# Autodesk Inventor assembly: VerticalParking
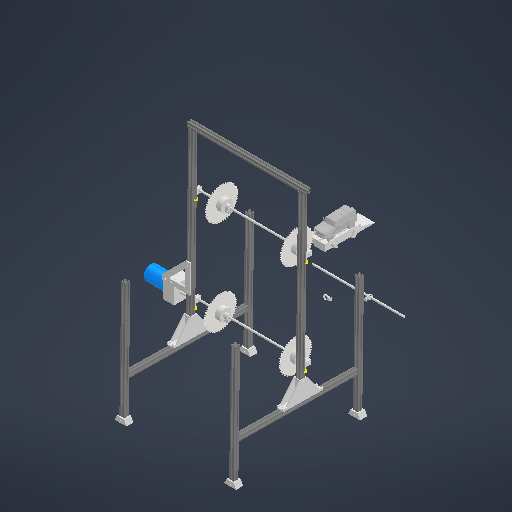
[picture p0: Inventor's stored thumbnail of the model, 512x512]
Saved by Autodesk Inventor 2026.1 (Build 301233020, 233B)
## iProperties
Created: 2025-12-07
Part Number: VerticalParking
Document SubType Name: Assembly
Designer: Tito Luyo Murata
Author: Tito Luyo Murata
## Documents named in this file (20)
- C:\work\verticalparking\diseno3d\VerticalParking.iam
- C:\work\verticalparking\diseno3d\01_Partes\soporte motor.ipt
- C:\work\verticalparking\diseno3d\01_Partes\Escuadra soporte motor.ipt
- C:\work\verticalparking\diseno3d\01_Partes\diseño piezas\motor_v02.ipt
- C:\work\verticalparking\diseno3d\01_Partes\Perfil_Aluminio_20x20x750.ipt
- C:\work\verticalparking\diseno3d\01_Partes\Perfil_Aluminio_20x20x500.ipt
- C:\work\verticalparking\diseno3d\01_Partes\base de soporte.ipt
- C:\work\verticalparking\diseno3d\01_Partes\SoportePrincipal.ipt
- C:\work\verticalparking\diseno3d\01_Partes\diseño piezas\soporte de eje de carril.ipt
- C:\work\verticalparking\diseno3d\01_Partes\diseño piezas\barrilla.ipt
- C:\work\verticalparking\diseno3d\01_Partes\diseño piezas\piñon.iam
- C:\work\verticalparking\diseno3d\01_Partes\SoporteEjePlato.ipt
- C:\work\verticalparking\diseno3d\01_Partes\SeguroRueda.ipt
- C:\work\verticalparking\diseno3d\01_Partes\RuedaDentada_v02.ipt
- C:\work\verticalparking\diseno3d\01_Partes\RuedaDentada_EjeFijo.ipt
- C:\work\verticalparking\diseno3d\01_Partes\Abrazadera.ipt
- C:\work\verticalparking\diseno3d\01_Partes\BaseCabina_v03.ipt
- C:\work\verticalparking\diseno3d\01_Partes\external\hammer_h3_v2\HermesH3v2.ipt
- C:\work\verticalparking\diseno3d\01_Partes\diseño piezas\barrilla_aluminio_385.ipt
- C:\work\verticalparking\diseno3d\01_Partes\AgarreColganteCabina_v02.ipt
## Components (55 placed, 19 different names)
1. soporte motor:1 — Mate:1, Mate:2, Mate:3, Mate:4, Mate:5, Mate:7
2. Escuadra soporte motor:1 — Mate:4, Mate:5, Mate:6, Mate:7, Flush:1, Flush:6
3. motor_v02:1 — Mate:1, Mate:2, Mate:3
4. Perfil_Aluminio_20x20x750:1 — Mate:9, Flush:3, Flush:5, Mate:16, Mate:17, Flush:16, Mate:18, Flush:17, Mate:29, Flush:21, Flush:23, Mate:32, Flush:26
5. Perfil_Aluminio_20x20x750:2 — Mate:6, Flush:1, Mate:8, Flush:2, Flush:4, Flush:6, Mate:14, Mate:15, Flush:15, Mate:19, Flush:19, Mate:30, Flush:22, Flush:24, Mate:33, Flush:27
6. Perfil_Aluminio_20x20x500:1 — Mate:8, Flush:2, Mate:9, Flush:3, Flush:4, Flush:5
7. Perfil_Aluminio_20x20x500:3 — Mate:10, Flush:7, Flush:8, Mate:11, Flush:9, Flush:10, Mate:18, Flush:17, Flush:18
8. Perfil_Aluminio_20x20x500:4 — Mate:11, Flush:9, Flush:10, Mate:26, Mate:27, Mate:28
9. Perfil_Aluminio_20x20x500:5 — Mate:12, Flush:11, Flush:12, Mate:20, Mate:21, Mate:22
10. Perfil_Aluminio_20x20x500:6 — Mate:13, Flush:13, Flush:14, Mate:23, Mate:24, Mate:25
11. Perfil_Aluminio_20x20x500:7 — Mate:10, Flush:7, Flush:8, Mate:51, Mate:52, Mate:53
12. Perfil_Aluminio_20x20x500:8 — Mate:12, Flush:11, Flush:12, Mate:13, Flush:13, Flush:14, Mate:19, Flush:19, Flush:20
13. base de soporte:1 — Mate:51, Mate:52, Mate:53
14. base de soporte:2 — Mate:23, Mate:24, Mate:25
15. base de soporte:3 — Mate:26, Mate:27, Mate:28
16. base de soporte:4 — Mate:20, Mate:21, Mate:22
17. SoportePrincipal:1 — Mate:16, Mate:17, Flush:16, Flush:18
18. SoportePrincipal:2 — Mate:14, Mate:15, Flush:15, Flush:20, Mate:74
19. soporte de eje de carril:1 — Mate:29, Flush:21, Flush:23, Mate:31, Flush:25
20. soporte de eje de carril:2 — Mate:30, Flush:22, Flush:24
21. barrilla:1 — Mate:31, Flush:25, Mate:38, Mate:39, Mate:63, Mate:65, Mate:70, Mate:71, Mate:72, Mate:73, Mate:87, Mate:88, Mate:89, Mate:90
22. soporte de eje de carril:3 — Mate:33, Flush:27, Mate:35, Mate:74
23. soporte de eje de carril:4 — Mate:32, Flush:26, Mate:34, Flush:28, Mate:91
24. barrilla:2 — Mate:34, Mate:35, Flush:28, Mate:36, Mate:37, Mate:40, Mate:44, Mate:46, Mate:49, Mate:55, Mate:57, Mate:59, Mate:61, Mate:76, Mate:80, Mate:81, Mate:82
25. piñon:1 [sub-assembly] — Mate:36, Mate:43, Mate:56, Mate:58, Flush:29
26. piñon:2 [sub-assembly] — Mate:37, Mate:42, Mate:54, Mate:60, Flush:30
27. piñon:3 [sub-assembly] — Mate:39, Mate:62, Mate:67, Mate:68, Flush:30
28. piñon:4 [sub-assembly] — Mate:38, Mate:64, Mate:66, Mate:69, Flush:29
29. SoporteEjePlato:1 — Mate:45, Mate:46, Mate:47
30. SoporteEjePlato:2 — Mate:48, Mate:49, Mate:50
31. SeguroRueda:1 — Mate:68, Mate:73, Mate:83
32. SeguroRueda:2 — Mate:69, Mate:70, Mate:84
33. SeguroRueda:3 — Mate:67, Mate:72, Mate:86
34. SeguroRueda:4 — Mate:66, Mate:71, Mate:85
35. SeguroRueda:5 — Mate:60, Mate:61, Mate:78
36. SeguroRueda:6 — Mate:58, Mate:59, Mate:77
37. SeguroRueda:7 — Mate:54, Mate:55, Mate:75
38. SeguroRueda:8 — Mate:56, Mate:57, Mate:79
39. RuedaDentada_v02:1 — Mate:62, Mate:63
40. RuedaDentada_v02:2 — Mate:64, Mate:65
41. RuedaDentada_EjeFijo:1 — Mate:40, Mate:42, Mate:48, Mate:50
42. RuedaDentada_EjeFijo:2 — Mate:43, Mate:44, Mate:45, Mate:47
43. Abrazadera:1 — Mate:75, Mate:76, Mate:91
44. Abrazadera:2 — Mate:83, Mate:88
45. Abrazadera:3 — Mate:84, Mate:89
46. Abrazadera:4 — Mate:79, Mate:80
47. Abrazadera:5 — Mate:77, Mate:81, Mate:92
48. Abrazadera:6 — Mate:78, Mate:82, Mate:92
49. Abrazadera:7 — Mate:86, Mate:87
50. Abrazadera:8 — Mate:85, Mate:90
51. BaseCabina_v03:1 — Mate:93
52. HermesH3v2:1 — Mate:93
53. barrilla_aluminio_385:1 — Mate:94
54. AgarreColganteCabina_v02:1 — Mate:94
55. AgarreColganteCabina_v02:2
## Relationships (123: Mate 93, Flush 30)
- Mate:1: soporte motor:1 ↔ motor_v02:1
- Mate:2: soporte motor:1 ↔ motor_v02:1
- Mate:3: soporte motor:1 ↔ motor_v02:1
- Mate:4: soporte motor:1 ↔ Escuadra soporte motor:1
- Mate:5: soporte motor:1 ↔ Escuadra soporte motor:1
- Mate:6: Escuadra soporte motor:1 ↔ Perfil_Aluminio_20x20x750:2
- Mate:7: soporte motor:1 ↔ Escuadra soporte motor:1
- Flush:1: Escuadra soporte motor:1 ↔ Perfil_Aluminio_20x20x750:2
- Mate:8: Perfil_Aluminio_20x20x750:2 ↔ Perfil_Aluminio_20x20x500:1
- Flush:2: Perfil_Aluminio_20x20x750:2 ↔ Perfil_Aluminio_20x20x500:1
- Mate:9: Perfil_Aluminio_20x20x750:1 ↔ Perfil_Aluminio_20x20x500:1
- Flush:3: Perfil_Aluminio_20x20x750:1 ↔ Perfil_Aluminio_20x20x500:1
- Flush:4 (-6.54 mm): Perfil_Aluminio_20x20x750:2 ↔ Perfil_Aluminio_20x20x500:1
- Flush:5 (12.92 mm): Perfil_Aluminio_20x20x750:1 ↔ Perfil_Aluminio_20x20x500:1
- Flush:6 (157 mm): Escuadra soporte motor:1 ↔ Perfil_Aluminio_20x20x750:2
- Mate:10: Perfil_Aluminio_20x20x500:3 ↔ Perfil_Aluminio_20x20x500:7
- Flush:7: Perfil_Aluminio_20x20x500:3 ↔ Perfil_Aluminio_20x20x500:7
- Flush:8 (150 mm): Perfil_Aluminio_20x20x500:3 ↔ Perfil_Aluminio_20x20x500:7
- Mate:11: Perfil_Aluminio_20x20x500:3 ↔ Perfil_Aluminio_20x20x500:4
- Flush:9: Perfil_Aluminio_20x20x500:3 ↔ Perfil_Aluminio_20x20x500:4
- Flush:10 (-150 mm): Perfil_Aluminio_20x20x500:3 ↔ Perfil_Aluminio_20x20x500:4
- Mate:12: Perfil_Aluminio_20x20x500:5 ↔ Perfil_Aluminio_20x20x500:8
- Flush:11: Perfil_Aluminio_20x20x500:5 ↔ Perfil_Aluminio_20x20x500:8
- Flush:12 (150 mm): Perfil_Aluminio_20x20x500:5 ↔ Perfil_Aluminio_20x20x500:8
- Mate:13: Perfil_Aluminio_20x20x500:6 ↔ Perfil_Aluminio_20x20x500:8
- Flush:13: Perfil_Aluminio_20x20x500:6 ↔ Perfil_Aluminio_20x20x500:8
- Flush:14 (150 mm): Perfil_Aluminio_20x20x500:6 ↔ Perfil_Aluminio_20x20x500:8
- Mate:14: Perfil_Aluminio_20x20x750:2 ↔ SoportePrincipal:2
- Mate:15: Perfil_Aluminio_20x20x750:2 ↔ SoportePrincipal:2
- Flush:15: Perfil_Aluminio_20x20x750:2 ↔ SoportePrincipal:2
- Mate:16: Perfil_Aluminio_20x20x750:1 ↔ SoportePrincipal:1
- Mate:17: Perfil_Aluminio_20x20x750:1 ↔ SoportePrincipal:1
- Flush:16: Perfil_Aluminio_20x20x750:1 ↔ SoportePrincipal:1
- Mate:18: Perfil_Aluminio_20x20x750:1 ↔ Perfil_Aluminio_20x20x500:3
- Flush:17: Perfil_Aluminio_20x20x750:1 ↔ Perfil_Aluminio_20x20x500:3
- Flush:18 (150 mm): Perfil_Aluminio_20x20x500:3 ↔ SoportePrincipal:1
- Mate:19: Perfil_Aluminio_20x20x750:2 ↔ Perfil_Aluminio_20x20x500:8
- Flush:19: Perfil_Aluminio_20x20x750:2 ↔ Perfil_Aluminio_20x20x500:8
- Flush:20 (150 mm): Perfil_Aluminio_20x20x500:8 ↔ SoportePrincipal:2
- Mate:20: Perfil_Aluminio_20x20x500:5 ↔ base de soporte:4
- Mate:21: Perfil_Aluminio_20x20x500:5 ↔ base de soporte:4
- Mate:22: Perfil_Aluminio_20x20x500:5 ↔ base de soporte:4
- Mate:23: Perfil_Aluminio_20x20x500:6 ↔ base de soporte:2
- Mate:24: Perfil_Aluminio_20x20x500:6 ↔ base de soporte:2
- Mate:25: Perfil_Aluminio_20x20x500:6 ↔ base de soporte:2
- Mate:26: Perfil_Aluminio_20x20x500:4 ↔ base de soporte:3
- Mate:27: Perfil_Aluminio_20x20x500:4 ↔ base de soporte:3
- Mate:28: Perfil_Aluminio_20x20x500:4 ↔ base de soporte:3
- Mate:29: Perfil_Aluminio_20x20x750:1 ↔ soporte de eje de carril:1
- Flush:21 (2.5 mm): Perfil_Aluminio_20x20x750:1 ↔ soporte de eje de carril:1
- Mate:30: Perfil_Aluminio_20x20x750:2 ↔ soporte de eje de carril:2
- Flush:22 (-2.5 mm): Perfil_Aluminio_20x20x750:2 ↔ soporte de eje de carril:2
- Flush:23 (215 mm): Perfil_Aluminio_20x20x750:1 ↔ soporte de eje de carril:1
- Flush:24 (215 mm): Perfil_Aluminio_20x20x750:2 ↔ soporte de eje de carril:2
- Mate:31: soporte de eje de carril:1 ↔ barrilla:1
- Flush:25 (5.5 mm): soporte de eje de carril:1 ↔ barrilla:1
- Mate:32: Perfil_Aluminio_20x20x750:1 ↔ soporte de eje de carril:4
- Flush:26 (2.5 mm): Perfil_Aluminio_20x20x750:1 ↔ soporte de eje de carril:4
- Mate:33: Perfil_Aluminio_20x20x750:2 ↔ soporte de eje de carril:3
- Flush:27 (2.5 mm): Perfil_Aluminio_20x20x750:2 ↔ soporte de eje de carril:3
- Mate:34: soporte de eje de carril:4 ↔ barrilla:2
- Mate:35: soporte de eje de carril:3 ↔ barrilla:2
- Flush:28 (-5.5 mm): soporte de eje de carril:4 ↔ barrilla:2
- Mate:36: barrilla:2 ↔ piñon:1
- Mate:37: barrilla:2 ↔ piñon:2
- Mate:38: barrilla:1 ↔ piñon:4
- Mate:39: barrilla:1 ↔ piñon:3
- Mate:40: barrilla:2 ↔ RuedaDentada_EjeFijo:1
- Mate:42: piñon:2 ↔ RuedaDentada_EjeFijo:1
- Mate:43: piñon:1 ↔ RuedaDentada_EjeFijo:2
- Mate:44: barrilla:2 ↔ RuedaDentada_EjeFijo:2
- Mate:45: SoporteEjePlato:1 ↔ RuedaDentada_EjeFijo:2
- Mate:46: barrilla:2 ↔ SoporteEjePlato:1
- Mate:47: SoporteEjePlato:1 ↔ RuedaDentada_EjeFijo:2
- Mate:48: SoporteEjePlato:2 ↔ RuedaDentada_EjeFijo:1
- Mate:49: barrilla:2 ↔ SoporteEjePlato:2
- Mate:50: SoporteEjePlato:2 ↔ RuedaDentada_EjeFijo:1
- Mate:51: Perfil_Aluminio_20x20x500:7 ↔ base de soporte:1
- Mate:52: Perfil_Aluminio_20x20x500:7 ↔ base de soporte:1
- Mate:53: Perfil_Aluminio_20x20x500:7 ↔ base de soporte:1
- Mate:54: piñon:2 ↔ SeguroRueda:7
- Mate:55: barrilla:2 ↔ SeguroRueda:7
- Mate:56: piñon:1 ↔ SeguroRueda:8
- Mate:57: barrilla:2 ↔ SeguroRueda:8
- Mate:58: piñon:1 ↔ SeguroRueda:6
- Mate:59: barrilla:2 ↔ SeguroRueda:6
- Mate:60: piñon:2 ↔ SeguroRueda:5
- Mate:61: barrilla:2 ↔ SeguroRueda:5
- Mate:62: piñon:3 ↔ RuedaDentada_v02:1
- Mate:63: barrilla:1 ↔ RuedaDentada_v02:1
- Mate:64: piñon:4 ↔ RuedaDentada_v02:2
- Mate:65: barrilla:1 ↔ RuedaDentada_v02:2
- Mate:66: piñon:4 ↔ SeguroRueda:4
- Mate:67: piñon:3 ↔ SeguroRueda:3
- Mate:68: piñon:3 ↔ SeguroRueda:1
- Mate:69: piñon:4 ↔ SeguroRueda:2
- Mate:70: barrilla:1 ↔ SeguroRueda:2
- Mate:71: barrilla:1 ↔ SeguroRueda:4
- Mate:72: barrilla:1 ↔ SeguroRueda:3
- Mate:73: barrilla:1 ↔ SeguroRueda:1
- Mate:74 (19.7 mm): SoportePrincipal:2 ↔ soporte de eje de carril:3
- Flush:29: piñon:1 ↔ piñon:4
- Flush:30: piñon:2 ↔ piñon:3
- Mate:75: SeguroRueda:7 ↔ Abrazadera:1
- Mate:76: barrilla:2 ↔ Abrazadera:1
- Mate:77: SeguroRueda:6 ↔ Abrazadera:5
- Mate:78: SeguroRueda:5 ↔ Abrazadera:6
- Mate:79: SeguroRueda:8 ↔ Abrazadera:4
- Mate:80: barrilla:2 ↔ Abrazadera:4
- Mate:81: barrilla:2 ↔ Abrazadera:5
- Mate:82: barrilla:2 ↔ Abrazadera:6
- Mate:83: SeguroRueda:1 ↔ Abrazadera:2
- Mate:84: SeguroRueda:2 ↔ Abrazadera:3
- Mate:85: SeguroRueda:4 ↔ Abrazadera:8
- Mate:86: SeguroRueda:3 ↔ Abrazadera:7
- Mate:87: barrilla:1 ↔ Abrazadera:7
- Mate:88: barrilla:1 ↔ Abrazadera:2
- Mate:89: barrilla:1 ↔ Abrazadera:3
- Mate:90: barrilla:1 ↔ Abrazadera:8
- Mate:91 (5 mm): soporte de eje de carril:4 ↔ Abrazadera:1
- Mate:92 (240 mm): Abrazadera:5 ↔ Abrazadera:6
- Mate:93: BaseCabina_v03:1 ↔ HermesH3v2:1
- Mate:94: barrilla_aluminio_385:1 ↔ AgarreColganteCabina_v02:1
